# Autodesk Inventor assembly: Configuration 1
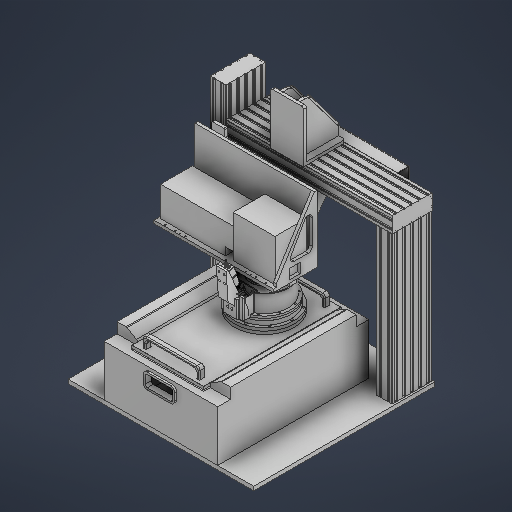
[picture p0: Inventor's stored thumbnail of the model, 512x512]
Saved by Autodesk Inventor 2026 (Build 300175000, 175)
## iProperties
Created: 2024-06-05
Part Number: Configuration 1
Document SubType Name: Assembly
Designer: AdminForWorker
Title: Printer Assembly v13
Author: AdminForWorker
## Documents named in this file (6)
- C:\School\Research\Inventor\v0.3\Printer\Printer Assembly.iam
- C:\School\Research\Inventor\v0.3\Printer\Laser w_ silver v4.iam
- C:\School\Research\Inventor\v0.3\Printer\Printer Body v6.ipt
- C:\School\Research\Inventor\v0.3\Printer\moving inner chamber piece v1 v2.ipt
- C:\School\Research\Inventor\v0.3\Printer\Printer Frame.ipt
- C:\School\Research\Inventor\v0.3\ASM\Cover Event Camera_PrinterPlate.iam
## Components (5 placed, 5 different names)
1. Laser w/ silver v4:1 [sub-assembly]
2. Printer Body v6:1 — Mate:1, Mate:2
3. moving inner chamber piece v1 v2:1
4. Cover Event Camera_PrinterPlate:1 [sub-assembly] — Mate:1, Mate:2
5. Part14
## Relationships (2: Mate 2)
- Mate:1: Printer Body v6:1 ↔ Cover Event Camera_PrinterPlate:1
- Mate:2: Printer Body v6:1 ↔ Cover Event Camera_PrinterPlate:1
